# Autodesk Inventor assembly: robotic_arm
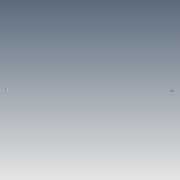
[picture p0: Inventor's stored thumbnail of the model, 180x180]
Saved by Autodesk Inventor 2013 (Build 170138000, 138)
## iProperties
Created: 2013-01-27
Part Number: robotic_arm
Document SubType Name: Assembly
Designer: idle-rug
Author: idle-rug
## Documents named in this file (14)
- C:\Users\Petr\Documents\Inventor\robotic arm\robotic_arm.iam
- C:\Users\Petr\Documents\Inventor\robotic arm\otocny_kruh.ipt
- C:\Users\Petr\Documents\Inventor\robotic arm\standart_servo.ipt
- C:\Users\Petr\Documents\Inventor\robotic arm\servo_paka1.ipt
- C:\Users\Petr\Documents\Inventor\robotic arm\servodrzak1.ipt
- C:\Users\Petr\Documents\Inventor\robotic arm\servodrzak0.ipt
- C:\Users\Petr\Documents\Inventor\robotic arm\stojan_cast1.ipt
- C:\Users\Petr\Documents\Inventor\robotic arm\loziskovy_uchyt.ipt
- C:\Users\Petr\Documents\Inventor\robotic arm\hridelka.ipt
- C:\Users\Petr\Documents\Inventor\robotic arm\dibond2.ipt
- C:\Users\Petr\Documents\Inventor\robotic arm\komatex.ipt
- C:\Users\Petr\Documents\Inventor\robotic arm\dibond3.ipt
- C:\Users\Petr\Documents\Inventor\robotic arm\ruka_backup.iam
- C:\Users\Petr\Documents\Inventor\robotic arm\micro_servo.ipt
## Components (25 placed, 13 different names)
1. otocny_kruh:1 — Mate:23, Mate:27, Mate:28, Mate:110
2. standart_servo:1 — Mate:2, Mate:3, Mate:6, Mate:7, Mate:8, Mate:20, Mate:21, Mate:22, Mate:44
3. servo_paka1:1 — Mate:2, Mate:3, Mate:45
4. servodrzak1:1 — Mate:6, Mate:7, Mate:8, Mate:23
5. servodrzak0:1 — Mate:20, Mate:21, Mate:22
6. stojan_cast1:1 — Mate:27, Mate:30, Mate:35
7. stojan_cast1:2 — Mate:28, Mate:30, Mate:33, Mate:34, Mate:51, Mate:83
8. loziskovy_uchyt:1 — Mate:83
9. hridelka:1 — Mate:35, Mate:44, Mate:45, Mate:51
10. dibond2:2 — Mate:57, Mate:58, Mate:88, Mate:98, Mate:99
11. standart_servo:2 — Mate:55, Mate:56
12. servo_paka1:2 — Mate:55, Mate:56, Mate:57, Mate:58
13. loziskovy_uchyt:2 — Mate:85, Mate:86, Mate:87
14. hridelka:2 — Mate:93
15. dibond2:3 — Mate:85, Mate:86, Mate:87, Mate:88, Mate:103, Mate:104, Mate:106, Mate:107, Mate:108, Mate:109
16. komatex:1 — Mate:93
17. dibond3:1 — Mate:96, Mate:97, Flush:1, Mate:105
18. dibond3:2 — Mate:100, Mate:101, Mate:102, Mate:105
19. standart_servo:3 — Mate:94, Mate:95, Mate:96, Flush:1
20. servo_paka1:3 — Mate:94, Mate:95, Mate:97, Mate:98, Mate:99
21. loziskovy_uchyt:3 — Mate:100, Mate:101, Mate:102, Mate:103, Mate:104
22. komatex:2 — Mate:107, Mate:108, Mate:109
23. hridelka:3 — Mate:106
24. ruka_backup:1 [sub-assembly] — Mate:110, Mate:111, Mate:112
25. micro_servo:1 — Mate:111, Mate:112
## Relationships (48: Mate 47, Flush 1)
- Mate:2: standart_servo:1 ↔ servo_paka1:1
- Mate:3: standart_servo:1 ↔ servo_paka1:1
- Mate:6: standart_servo:1 ↔ servodrzak1:1
- Mate:7: standart_servo:1 ↔ servodrzak1:1
- Mate:8: standart_servo:1 ↔ servodrzak1:1
- Mate:20: standart_servo:1 ↔ servodrzak0:1
- Mate:21: standart_servo:1 ↔ servodrzak0:1
- Mate:22: standart_servo:1 ↔ servodrzak0:1
- Mate:23: otocny_kruh:1 ↔ servodrzak1:1
- Mate:27: otocny_kruh:1 ↔ stojan_cast1:1
- Mate:28: otocny_kruh:1 ↔ stojan_cast1:2
- Mate:30: stojan_cast1:1 ↔ stojan_cast1:2
- Mate:33: stojan_cast1:2
- Mate:34 (8 mm): stojan_cast1:2
- Mate:35: stojan_cast1:1 ↔ hridelka:1
- Mate:44: standart_servo:1 ↔ hridelka:1
- Mate:45: servo_paka1:1 ↔ hridelka:1
- Mate:51: stojan_cast1:2 ↔ hridelka:1
- Mate:55: standart_servo:2 ↔ servo_paka1:2
- Mate:56: standart_servo:2 ↔ servo_paka1:2
- Mate:57: dibond2:2 ↔ servo_paka1:2
- Mate:58: dibond2:2 ↔ servo_paka1:2
- Mate:83 (0.5 mm): stojan_cast1:2 ↔ loziskovy_uchyt:1
- Mate:85: loziskovy_uchyt:2 ↔ dibond2:3
- Mate:86: loziskovy_uchyt:2 ↔ dibond2:3
- Mate:87: loziskovy_uchyt:2 ↔ dibond2:3
- Mate:88: dibond2:2 ↔ dibond2:3
- Mate:93: hridelka:2 ↔ komatex:1
- Mate:94: standart_servo:3 ↔ servo_paka1:3
- Mate:95: standart_servo:3 ↔ servo_paka1:3
- Mate:96: dibond3:1 ↔ standart_servo:3
- Mate:97: dibond3:1 ↔ servo_paka1:3
- Flush:1: dibond3:1 ↔ standart_servo:3
- Mate:98: dibond2:2 ↔ servo_paka1:3
- Mate:99: dibond2:2 ↔ servo_paka1:3
- Mate:100: dibond3:2 ↔ loziskovy_uchyt:3
- Mate:101: dibond3:2 ↔ loziskovy_uchyt:3
- Mate:102: dibond3:2 ↔ loziskovy_uchyt:3
- Mate:103: dibond2:3 ↔ loziskovy_uchyt:3
- Mate:104 (0.5 mm): dibond2:3 ↔ loziskovy_uchyt:3
- Mate:105: dibond3:1 ↔ dibond3:2
- Mate:106: dibond2:3 ↔ hridelka:3
- Mate:107: dibond2:3 ↔ komatex:2
- Mate:108: dibond2:3 ↔ komatex:2
- Mate:109: dibond2:3 ↔ komatex:2
- Mate:110: otocny_kruh:1 ↔ ruka_backup:1
- Mate:111: ruka_backup:1 ↔ micro_servo:1
- Mate:112: ruka_backup:1 ↔ micro_servo:1
